# Autodesk Inventor assembly: Panel A
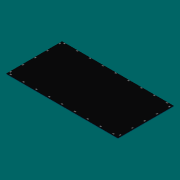
[picture p0: Inventor's stored thumbnail of the model, 180x180]
Saved by Autodesk Inventor 2016 (Build 200138000, 138)
## iProperties
Created: 2015-06-04
Part Number: Panel A
Document SubType Name: Assembly
Designer: Sawaiz Syed
Author: Sawaiz Syed
## Documents named in this file (4)
- C:\Users\Sawaiz\Documents\data\projects\cncBlackBox\panels\panelA.iam
- C:\Users\Sawaiz\Documents\data\projects\cncBlackBox\panels\faceA.ipt
- C:\Users\Sawaiz\Documents\data\projects\cncBlackBox\panels\faceAFelt.ipt
- C:\Users\Sawaiz\Documents\data\projects\cncBlackBox\panels\facingScrew.iam
## Components (30 placed, 3 different names)
1. faceA:1 — Mate:1, Mate:2, Mate:3, Mate:4, Mate:5, Angle:1, Mate:6, Angle:2, Mate:7, Mate:8
2. faceAFelt:1 — Mate:1, Mate:2, Mate:3
3. facingScrew:1 [sub-assembly] — Mate:4, Mate:5, Angle:1, Mate:8
4. facingScrew:2 [sub-assembly]
5. facingScrew:3 [sub-assembly]
6. facingScrew:4 [sub-assembly]
7. facingScrew:5 [sub-assembly]
8. facingScrew:6 [sub-assembly]
9. facingScrew:7 [sub-assembly]
10. facingScrew:8 [sub-assembly]
11. facingScrew:9 [sub-assembly]
12. facingScrew:10 [sub-assembly]
13. facingScrew:11 [sub-assembly]
14. facingScrew:12 [sub-assembly]
15. facingScrew:13 [sub-assembly]
16. facingScrew:14 [sub-assembly]
17. facingScrew:15 [sub-assembly]
18. facingScrew:16 [sub-assembly]
19. facingScrew:17 [sub-assembly]
20. facingScrew:18 [sub-assembly]
21. facingScrew:19 [sub-assembly] — Mate:6, Angle:2, Mate:7
22. facingScrew:20 [sub-assembly]
23. facingScrew:21 [sub-assembly]
24. facingScrew:22 [sub-assembly]
25. facingScrew:23 [sub-assembly]
26. facingScrew:24 [sub-assembly]
27. facingScrew:25 [sub-assembly]
28. facingScrew:26 [sub-assembly]
29. facingScrew:27 [sub-assembly]
30. facingScrew:28 [sub-assembly]
## Component patterns: (18 elements, first: facingScrew:1), (10 elements, first: facingScrew:19)
## Relationships (10: Mate 8, Angle 2)
- Mate:1: faceA:1 ↔ faceAFelt:1
- Mate:2: faceA:1 ↔ faceAFelt:1
- Mate:3: faceA:1 ↔ faceAFelt:1
- Mate:4: faceA:1 ↔ facingScrew:1
- Mate:5: faceA:1 ↔ facingScrew:1
- Angle:1 (0 deg): faceA:1 ↔ facingScrew:1
- Mate:6: faceA:1 ↔ facingScrew:19
- Angle:2 (0 deg): faceA:1 ↔ facingScrew:19
- Mate:7: faceA:1 ↔ facingScrew:19
- Mate:8: faceA:1 ↔ facingScrew:1
